# Autodesk Inventor assembly: iparts_assembly
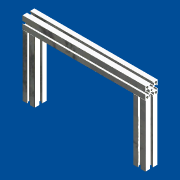
[picture p0: Inventor's stored thumbnail of the model, 180x180]
Saved by Autodesk Inventor 2022.2 (Build 262287000, 287)
## iProperties
Created: 2022-01-17
Part Number: iparts_assembly
Document SubType Name: Assembly
Designer: gisen
Author: gisen
## Documents named in this file (4)
- C:\Users\gisen\Desktop\iparts_test\iparts_assembly.iam
- C:\Users\gisen\Desktop\iparts_test\M4_almiflame\S100.ipt
- C:\Users\gisen\Desktop\iparts_test\M4_almiflame.ipt
- C:\Users\gisen\Desktop\iparts_test\M4_almiflame\S200.ipt
## Components (3 placed, 2 different names)
1. S100:1 — フラッシュ:1, メイト:1, フラッシュ:2
2. S200:2 — フラッシュ:1, メイト:1, フラッシュ:2, メイト:2, フラッシュ:3, フラッシュ:4
3. S100:3 — メイト:2, フラッシュ:3, フラッシュ:4
## Relationships (6: Flush 4, Mate 2)
- フラッシュ:1 [Flush]: S100:1 ↔ S200:2
- メイト:1 [Mate]: S100:1 ↔ S200:2
- フラッシュ:2 [Flush]: S100:1 ↔ S200:2
- メイト:2 [Mate]: S200:2 ↔ S100:3
- フラッシュ:3 [Flush]: S200:2 ↔ S100:3
- フラッシュ:4 [Flush]: S200:2 ↔ S100:3
